# Autodesk Inventor assembly: full_axis
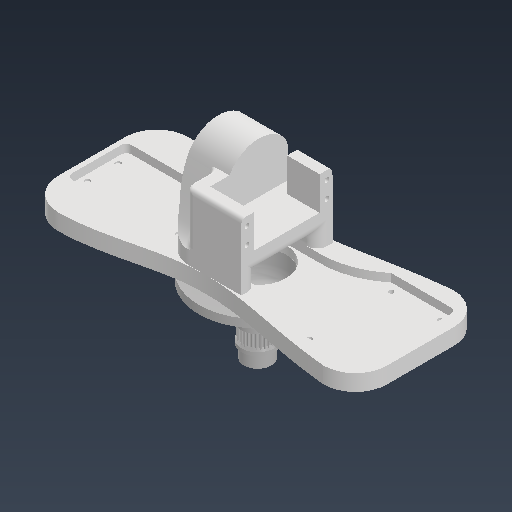
[picture p0: Inventor's stored thumbnail of the model, 512x512]
Saved by Autodesk Inventor 2026.1 (Build 301233020, 233B)
## iProperties
Created: 2025-12-02
Part Number: full_axis
Document SubType Name: Assembly
Designer: Piter
Author: Piter
## Documents named in this file (3)
- C:\Users\Piter\OneDrive\Pulpit\Robots\david_Arm\Davie-Robot-Arm\3D Models\full_axis.iam
- C:\Users\Piter\OneDrive\Pulpit\Robots\david_Arm\Davie-Robot-Arm\3D Models\Axis1_top_v2.ipt
- C:\Users\Piter\OneDrive\Pulpit\Robots\david_Arm\Davie-Robot-Arm\3D Models\Axis1_shaft_v2.ipt
## Components (2 placed, 2 different names)
1. Axis1_top_v2:1 — Rigid:1
2. Axis1_shaft_v2:1 — Rigid:1
## Relationships (1: WeldJoint 1)
- Rigid:1 [WeldJoint]: Axis1_top_v2:1 ↔ Axis1_shaft_v2:1
